# Autodesk Inventor assembly: 足ユニット
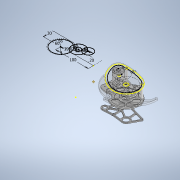
[picture p0: Inventor's stored thumbnail of the model, 180x180]
Saved by Autodesk Inventor 2022.2 (Build 262287010, 287A)
## iProperties
Created: 2022-01-10
Part Number: 足ユニット
Document SubType Name: Assembly
Designer: acps
Author: acps
## Documents named in this file (10)
- C:\Users\acps\Documents\srdc\srdc_ksh\足ユニット.iam
- C:\Users\acps\Documents\srdc\srdc_ksh\足(単独).iam
- C:\Users\acps\Documents\srdc\srdc_ksh\足外フレーム.ipt
- C:\Users\acps\Documents\srdc\srdc_ksh\足内フレーム.ipt
- C:\Users\acps\Documents\srdc\srdc_ksh\スペーサ\l40.ipt
- C:\Users\acps\Documents\srdc\srdc_ksh\カム\カム4.ipt
- C:\Users\acps\Documents\srdc\srdc_ksh\オイレス\w5f15-17n.ipt
- C:\Users\acps\Documents\srdc\srdc_ksh\モータ\M-RS-380.ipt
- C:\Users\acps\Documents\srdc\srdc_ksh\ギア抑え.ipt
- C:\Users\acps\Documents\srdc\srdc_ksh\モータマウント.ipt
## Components (11 placed, 9 different names)
1. 足外フレーム:1 — Insert:1, Mate:1, Insert:2, Insert:7
2. 足(単独):1 [sub-assembly] — Insert:1, Mate:1, Mate:2, Mate:3, Mate:5, Mate:6, Insert:6
3. 足内フレーム:1 — Mate:2, Mate:3, Mate:4, Insert:8, Mate:10, Mate:13, Mate:14, Mate:15, Insert:10
4. l40:1 — Insert:2
5. l40:2 — Insert:7, Insert:8
6. l40:3
7. カム4:1 — Mate:4, Mate:5, Mate:6, Insert:6, Insert:9
8. w5f15-17n:1 — Insert:9
9. M-RS-380:1 — Mate:10, Mate:16, Mate:17, Mate:18
10. ギア抑え:1 — Mate:13
11. モータマウント:1 — Mate:14, Mate:15, Insert:10, Mate:16, Mate:17, Mate:18
## Relationships (20: Mate 13, Insert 7)
- Insert:1 (0.5 mm): 足外フレーム:1 ↔ 足(単独):1
- Mate:1: 足外フレーム:1 ↔ 足(単独):1
- Mate:2: 足(単独):1 ↔ 足内フレーム:1
- Mate:3: 足(単独):1 ↔ 足内フレーム:1
- Insert:2: 足外フレーム:1 ↔ l40:1
- Mate:4: 足内フレーム:1 ↔ カム4:1
- Mate:5: 足(単独):1 ↔ カム4:1
- Mate:6: 足(単独):1 ↔ カム4:1
- Insert:6: 足(単独):1 ↔ カム4:1
- Insert:7: 足外フレーム:1 ↔ l40:2
- Insert:8: 足内フレーム:1 ↔ l40:2
- Insert:9: カム4:1 ↔ w5f15-17n:1
- Mate:10: 足内フレーム:1 ↔ M-RS-380:1
- Mate:13: 足内フレーム:1 ↔ ギア抑え:1
- Mate:14: 足内フレーム:1 ↔ モータマウント:1
- Mate:15: 足内フレーム:1 ↔ モータマウント:1
- Insert:10: 足内フレーム:1 ↔ モータマウント:1
- Mate:16: M-RS-380:1 ↔ モータマウント:1
- Mate:17: M-RS-380:1 ↔ モータマウント:1
- Mate:18: M-RS-380:1 ↔ モータマウント:1
